# Autodesk Inventor assembly: ArmTruss
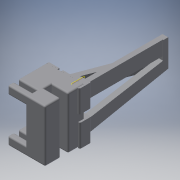
[picture p0: Inventor's stored thumbnail of the model, 180x180]
Saved by Autodesk Inventor 2018 (Build 220112000, 112)
## iProperties
Created: 2017-12-31
Part Number: ArmTruss
Document SubType Name: Assembly
Designer: reide
Author: reide
## Documents named in this file (5)
- C:\Users\reide\OneDrive\Documents\Inventor\TSA\2018\Animatronics\Tortoise\arms\ArmTruss.iam
- C:\Users\reide\OneDrive\Documents\Inventor\TSA\2018\Animatronics\Tortoise\arms\newShoulder.ipt
- C:\Users\reide\OneDrive\Documents\Inventor\TSA\2018\Animatronics\Tortoise\arms\straightBar.ipt
- C:\Users\reide\OneDrive\Documents\Inventor\TSA\2018\Animatronics\Tortoise\arms\AngleArm.ipt
- C:\Users\reide\OneDrive\Documents\Inventor\TSA\2018\Animatronics\Tortoise\arms\bottomARM.ipt
## Components (4 placed, 4 different names)
1. newShoulder:1
2. straightBar:1
3. AngleArm:1
4. bottomARM:1
## Relationships (9: Mate 5, Flush 4)
- [Flush]: newShoulder:1 ↔ AngleArm:1
- [Mate]: newShoulder:1 ↔ AngleArm:1
- [Mate]: newShoulder:1 ↔ AngleArm:1
- [Flush]: newShoulder:1 ↔ straightBar:1
- [Mate]: newShoulder:1 ↔ straightBar:1
- [Mate]: newShoulder:1 ↔ straightBar:1
- [Mate]: newShoulder:1 ↔ bottomARM:1
- [Flush]: newShoulder:1 ↔ bottomARM:1
- [Flush]: newShoulder:1 ↔ bottomARM:1
